# Autodesk Inventor assembly: Tension_Idler_A_Live
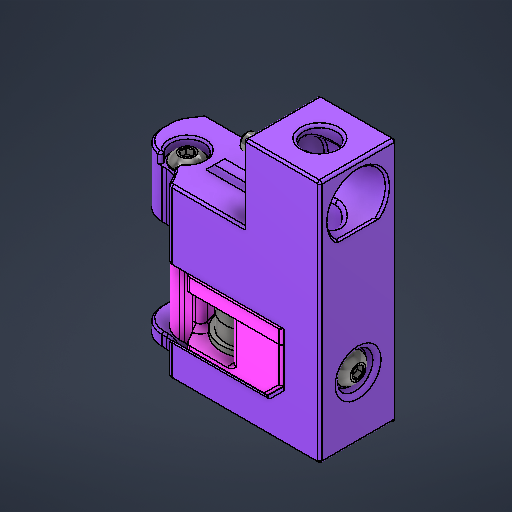
[picture p0: Inventor's stored thumbnail of the model, 512x512]
Saved by Autodesk Inventor 2026 (Build 300175050, 175E)
## iProperties
Created: 2025-05-26
Part Number: Tension_Idler_A_Live
Document SubType Name: Assembly
Designer: Joshua Eah
Author: Joshua Eah
## Documents named in this file (10)
- C:\Users\Joshua Eah\Documents\GitHub\Voron-0\CAD\Tulip - Machined Parts\V0.2R1 Tulip Mod Live Idlers v4\Tension_Idler_A_Live.iam
- C:\Users\Joshua Eah\Documents\GitHub\Voron-0\CAD\Tulip - Machined Parts\V0.2R1 Tulip Mod Live Idlers v4\Idler_A_Pin 3x18.ipt
- C:\Users\Joshua Eah\Documents\GitHub\Voron-0\CAD\Master Assembly\Hardware\F623 Stack.iam
- C:\Users\Joshua Eah\Documents\GitHub\Voron-0\CAD\Tulip - Machined Parts\V0.2R1 Tulip Mod Live Idlers v4\A_Idler_Static_x1.ipt
- C:\Users\Joshua Eah\Documents\GitHub\Voron-0\CAD\Tulip - Machined Parts\V0.2R1 Tulip Mod Live Idlers v4\[a]_Idler_A_Tensioner_Upper_x1.ipt
- C:\Users\Joshua Eah\Documents\GitHub\Voron-0\CAD\Tulip - Machined Parts\V0.2R1 Tulip Mod Live Idlers v4\[a]_Idler_A_Tensioner_Lower_x1.ipt
- C:\Users\Joshua Eah\Documents\GitHub\Voron-0\CAD\Master Assembly\Hardware\M3x10 BHCS.ipt
- C:\Users\Joshua Eah\Documents\GitHub\Voron-0\CAD\Master Assembly\Hardware\M3 Hexnut.ipt
- C:\Users\Joshua Eah\Documents\GitHub\Voron-0\CAD\Master Assembly\Hardware\M3x12 BHCS.ipt
- C:\Users\Joshua Eah\Documents\GitHub\Voron-0\CAD\Master Assembly\Hardware\M3x35 BHCS.ipt
## Components (10 placed, 9 different names)
1. A_Idler_Static_x1:1 — Insert:1, Insert:2, Insert:3, Insert:4
2. F623 Stack:1 [sub-assembly]
3. Idler_A_Pin 3x18:1
4. [a]_Idler_A_Tensioner_Upper_x1:1
5. [a]_Idler_A_Tensioner_Lower_x1:1
6. M3 Hexnut:2
7. M3x10 BHCS:2 — Insert:4
8. M3x10 BHCS:3 — Insert:2
9. M3x12 BHCS:2 — Insert:1
10. M3x35 BHCS:2 — Insert:3
## Relationships (4: Insert 4)
- Insert:1: A_Idler_Static_x1:1 ↔ M3x12 BHCS:2
- Insert:2: A_Idler_Static_x1:1 ↔ M3x10 BHCS:3
- Insert:3: A_Idler_Static_x1:1 ↔ M3x35 BHCS:2
- Insert:4: A_Idler_Static_x1:1 ↔ M3x10 BHCS:2
